# Autodesk Inventor assembly: ASY MSC 900.8 base frame transverse
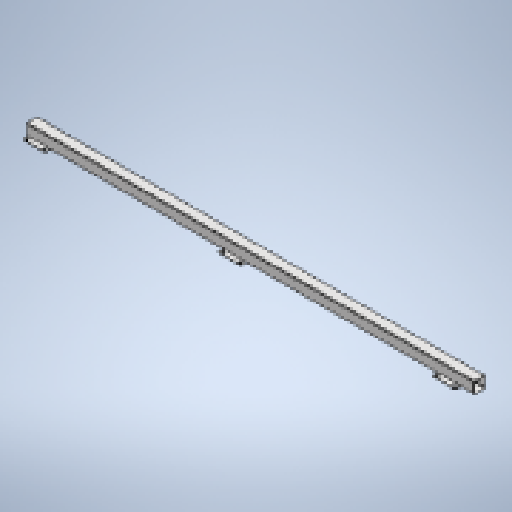
[picture p0: Inventor's stored thumbnail of the model, 512x512]
Saved by Autodesk Inventor 2025 (Build 290162010, 162A)
## iProperties
Created: 2024-09-07
Part Number: ASY MSC 900.8 base frame transverse
Document SubType Name: Assembly
Designer: pokla
Author: pokla
## Documents named in this file (3)
- C:\Users\user\YandexDisk-badmisterfox\домашниий пк\Inventor\Manturovo\Manturovo_Se-clar\ASY MSC 900.8 base frame transverse.iam
- C:\Users\user\YandexDisk-badmisterfox\домашниий пк\Inventor\Manturovo\Manturovo_Se-clar\MSC 908 transverse pillar plate.ipt
- C:\Users\user\YandexDisk-badmisterfox\домашниий пк\Inventor\Manturovo\Manturovo_Se-clar\ISO 4019 - 80x80x3 - 0,001.ipt
## Components (4 placed, 2 different names)
1. ASY MSC 900.8 base frame transverse:1 — Rigid:1
2. ASY MSC 900.8 base frame transverse:2 — Rigid:2, Rigid:3
3. ASY MSC 900.8 base frame transverse:3 — Rigid:3
4. ISO 4019 - 80x80x3 - 0,001:1 — Rigid:1, Rigid:2
## Relationships (3: WeldJoint 3)
- Rigid:1 [WeldJoint]: ASY MSC 900.8 base frame transverse:1 ↔ ISO 4019 - 80x80x3 - 0,001:1
- Rigid:2 [WeldJoint]: ASY MSC 900.8 base frame transverse:2 ↔ ISO 4019 - 80x80x3 - 0,001:1
- Rigid:3 [WeldJoint] (-1510 mm): ASY MSC 900.8 base frame transverse:2 ↔ ASY MSC 900.8 base frame transverse:3
